# Autodesk Inventor assembly: EL2-GB-100
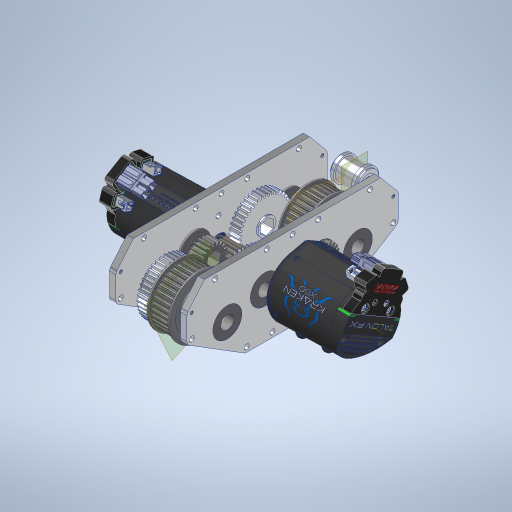
[picture p0: Inventor's stored thumbnail of the model, 512x512]
Saved by Autodesk Inventor 2023.4 (Build 274418000, 418)
## iProperties
Created: 2025-01-18
Part Number: EL2-GB-100
Document SubType Name: Assembly
Designer: jmcintyr
Author: jmcintyr
## Documents named in this file (10)
- C:\Users\jmcintyr\Documents\GitHub\2025-ReefScape---CAD\Elevator\EL2-GB\EL2-GB-100.iam
- C:\Users\jmcintyr\Documents\GitHub\2025-ReefScape---CAD\Elevator\EL2-GB\EL2-GB-001.ipt
- C:\Users\jmcintyr\Documents\GitHub\2025-ReefScape---CAD\Elevator\EL2-GB\EL2-GB-002.ipt
- C:\Users\jmcintyr\Documents\GitHub\2025-ReefScape---CAD\COMMON PARTS\MOTORS\Kracken with Cover and Boards.iam
- C:\Users\jmcintyr\Documents\GitHub\2025-ReefScape---CAD\COMMON PARTS\BEARINGS\0_500_ID_x_1_125_OD_x_0_313_WD_Flanged_Bearing_217-2731.ipt
- C:\Users\jmcintyr\Documents\GitHub\2025-ReefScape---CAD\COMMON PARTS\GEARS\20dp .5 hex\20t_Aluminum_Spur_Gear_20_DP_1_2_Hex_Bore_217-2702.ipt
- C:\Users\jmcintyr\Documents\GitHub\2025-ReefScape---CAD\COMMON PARTS\GEARS\12t 20 dp kracken WCP-1010.ipt
- C:\Users\jmcintyr\Documents\GitHub\2025-ReefScape---CAD\COMMON PARTS\GEARS\20dp .5 hex\40t_Aluminum_Spur_Gear_20_DP_1_2_Hex_Bore_217-2708.ipt
- C:\Users\jmcintyr\Documents\GitHub\2025-ReefScape---CAD\COMMON PARTS\PULLEYS\htd\36t_x_15mm_Wide_Aluminum_Pulley_HTD_5mm_1_2_Hex_217-4103.ipt
- C:\Users\jmcintyr\Documents\GitHub\2025-ReefScape---CAD\Elevator\EL2-GB\EL2-GB-200.iam
## Components (25 placed, 9 different names)
1. EL2-GB-001:1 — Insert:3, Insert:4, Insert:10, Insert:11, Insert:16, Insert:17, Insert:18, Insert:19, Mate:4, Symmetry:1, Mate:18
2. EL2-GB-001:2 — Insert:8, Insert:9, Insert:12, Insert:13, Insert:14, Insert:15, Mate:3, Symmetry:1
3. EL2-GB-002:1 — Insert:3
4. EL2-GB-002:5 — Insert:4
5. Kracken with Cover and Boards:1 [sub-assembly] — Insert:8, Insert:9, Mate:1
6. Kracken with Cover and Boards:2 [sub-assembly] — Insert:10, Insert:11, Mate:2
7. 0_500_ID_x_1_125_OD_x_0_313_WD_Flanged_Bearing_217-2731:1 — Insert:16, Mate:7
8. 0_500_ID_x_1_125_OD_x_0_313_WD_Flanged_Bearing_217-2731:2 — Insert:17
9. 0_500_ID_x_1_125_OD_x_0_313_WD_Flanged_Bearing_217-2731:3 — Insert:18, Mate:14
10. 0_500_ID_x_1_125_OD_x_0_313_WD_Flanged_Bearing_217-2731:4 — Insert:19, Mate:13
11. 0_500_ID_x_1_125_OD_x_0_313_WD_Flanged_Bearing_217-2731:5 — Insert:12, Mate:10
12. 0_500_ID_x_1_125_OD_x_0_313_WD_Flanged_Bearing_217-2731:6 — Insert:13, Mate:5, Mate:6
13. 0_500_ID_x_1_125_OD_x_0_313_WD_Flanged_Bearing_217-2731:7 — Insert:14, Mate:11
14. 0_500_ID_x_1_125_OD_x_0_313_WD_Flanged_Bearing_217-2731:8 — Insert:15
15. 20t_Aluminum_Spur_Gear_20_DP_1_2_Hex_Bore_217-2702:1 — Mate:6
16. 20t_Aluminum_Spur_Gear_20_DP_1_2_Hex_Bore_217-2702:2 — Mate:14
17. 12t 20 dp kracken WCP-1010:1 — Mate:1, Mate:3, Flush:3
18. 12t 20 dp kracken WCP-1010:2 — Mate:2, Mate:4, Flush:2
19. 40t_Aluminum_Spur_Gear_20_DP_1_2_Hex_Bore_217-2708:1 — Mate:11, Flush:3
20. 40t_Aluminum_Spur_Gear_20_DP_1_2_Hex_Bore_217-2708:2 — Mate:5, Flush:2
21. 40t_Aluminum_Spur_Gear_20_DP_1_2_Hex_Bore_217-2708:3 — Mate:7
22. 36t_x_15mm_Wide_Aluminum_Pulley_HTD_5mm_1_2_Hex_217-4103:1 — Mate:9, Mate:10, Mate:15
23. 40t_Aluminum_Spur_Gear_20_DP_1_2_Hex_Bore_217-2708:4 — Mate:13, Mate:16
24. 36t_x_15mm_Wide_Aluminum_Pulley_HTD_5mm_1_2_Hex_217-4103:2 — Mate:15, Mate:16, Mate:17
25. EL2-GB-200:1 [sub-assembly] — Mate:17, Mate:18
## Relationships (33: Mate 16, Insert 14, Flush 2, Symmetry 1)
- Insert:3: EL2-GB-001:1 ↔ EL2-GB-002:1
- Insert:4: EL2-GB-001:1 ↔ EL2-GB-002:5
- Insert:8: EL2-GB-001:2 ↔ Kracken with Cover and Boards:1
- Insert:9: EL2-GB-001:2 ↔ Kracken with Cover and Boards:1
- Insert:10: EL2-GB-001:1 ↔ Kracken with Cover and Boards:2
- Insert:11: EL2-GB-001:1 ↔ Kracken with Cover and Boards:2
- Insert:12: EL2-GB-001:2 ↔ 0_500_ID_x_1_125_OD_x_0_313_WD_Flanged_Bearing_217-2731:5
- Insert:13: EL2-GB-001:2 ↔ 0_500_ID_x_1_125_OD_x_0_313_WD_Flanged_Bearing_217-2731:6
- Insert:14: EL2-GB-001:2 ↔ 0_500_ID_x_1_125_OD_x_0_313_WD_Flanged_Bearing_217-2731:7
- Insert:15: EL2-GB-001:2 ↔ 0_500_ID_x_1_125_OD_x_0_313_WD_Flanged_Bearing_217-2731:8
- Insert:16: EL2-GB-001:1 ↔ 0_500_ID_x_1_125_OD_x_0_313_WD_Flanged_Bearing_217-2731:1
- Insert:17: EL2-GB-001:1 ↔ 0_500_ID_x_1_125_OD_x_0_313_WD_Flanged_Bearing_217-2731:2
- Insert:18: EL2-GB-001:1 ↔ 0_500_ID_x_1_125_OD_x_0_313_WD_Flanged_Bearing_217-2731:3
- Insert:19: EL2-GB-001:1 ↔ 0_500_ID_x_1_125_OD_x_0_313_WD_Flanged_Bearing_217-2731:4
- Mate:1: Kracken with Cover and Boards:1 ↔ 12t 20 dp kracken WCP-1010:1
- Mate:2: Kracken with Cover and Boards:2 ↔ 12t 20 dp kracken WCP-1010:2
- Mate:3 (3.175 mm): EL2-GB-001:2 ↔ 12t 20 dp kracken WCP-1010:1
- Mate:4 (3.175 mm): EL2-GB-001:1 ↔ 12t 20 dp kracken WCP-1010:2
- Mate:5: 0_500_ID_x_1_125_OD_x_0_313_WD_Flanged_Bearing_217-2731:6 ↔ 40t_Aluminum_Spur_Gear_20_DP_1_2_Hex_Bore_217-2708:2
- Mate:6: 0_500_ID_x_1_125_OD_x_0_313_WD_Flanged_Bearing_217-2731:6 ↔ 20t_Aluminum_Spur_Gear_20_DP_1_2_Hex_Bore_217-2702:1
- Mate:7: 0_500_ID_x_1_125_OD_x_0_313_WD_Flanged_Bearing_217-2731:1 ↔ 40t_Aluminum_Spur_Gear_20_DP_1_2_Hex_Bore_217-2708:3
- Flush:2: 12t 20 dp kracken WCP-1010:2 ↔ 40t_Aluminum_Spur_Gear_20_DP_1_2_Hex_Bore_217-2708:2
- Symmetry:1: EL2-GB-001:1 ↔ EL2-GB-001:2
- Mate:9: 36t_x_15mm_Wide_Aluminum_Pulley_HTD_5mm_1_2_Hex_217-4103:1
- Mate:10: 0_500_ID_x_1_125_OD_x_0_313_WD_Flanged_Bearing_217-2731:5 ↔ 36t_x_15mm_Wide_Aluminum_Pulley_HTD_5mm_1_2_Hex_217-4103:1
- Mate:11: 0_500_ID_x_1_125_OD_x_0_313_WD_Flanged_Bearing_217-2731:7 ↔ 40t_Aluminum_Spur_Gear_20_DP_1_2_Hex_Bore_217-2708:1
- Mate:13: 0_500_ID_x_1_125_OD_x_0_313_WD_Flanged_Bearing_217-2731:4 ↔ 40t_Aluminum_Spur_Gear_20_DP_1_2_Hex_Bore_217-2708:4
- Flush:3 (3.175 mm): 12t 20 dp kracken WCP-1010:1 ↔ 40t_Aluminum_Spur_Gear_20_DP_1_2_Hex_Bore_217-2708:1
- Mate:14: 0_500_ID_x_1_125_OD_x_0_313_WD_Flanged_Bearing_217-2731:3 ↔ 20t_Aluminum_Spur_Gear_20_DP_1_2_Hex_Bore_217-2702:2
- Mate:15: 36t_x_15mm_Wide_Aluminum_Pulley_HTD_5mm_1_2_Hex_217-4103:1 ↔ 36t_x_15mm_Wide_Aluminum_Pulley_HTD_5mm_1_2_Hex_217-4103:2
- Mate:16: 40t_Aluminum_Spur_Gear_20_DP_1_2_Hex_Bore_217-2708:4 ↔ 36t_x_15mm_Wide_Aluminum_Pulley_HTD_5mm_1_2_Hex_217-4103:2
- Mate:17: 36t_x_15mm_Wide_Aluminum_Pulley_HTD_5mm_1_2_Hex_217-4103:2 ↔ EL2-GB-200:1
- Mate:18: EL2-GB-001:1 ↔ EL2-GB-200:1
